# Autodesk Inventor assembly: GFRP_T2_18
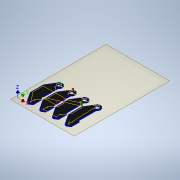
[picture p0: Inventor's stored thumbnail of the model, 180x180]
Saved by Autodesk Inventor 2020 (Build 240168000, 168)
## iProperties
Created: 2021-08-27
Part Number: GFRP_T2_18
Document SubType Name: Assembly
Designer: Masato
Author: Masato
## Documents named in this file (3)
- D:\GitHub\inventor\SUSTAINA-OP\Cam\GFRP_T2_18.iam
- D:\GitHub\inventor\SUSTAINA-OP\Cam\DisposableBoard.ipt
- D:\GitHub\inventor\SUSTAINA-OP\LowerBody\Link\FrontLink_frame.ipt
## Components (5 placed, 2 different names)
1. DisposableBoard:1 — メイト:2, メイト:1, フラッシュ:1, フラッシュ:2, メイト:6, メイト:7, 正接:2
2. FrontLink_frame:1 — メイト:6, メイト:7, 正接:2
3. FrontLink_frame:2
4. FrontLink_frame:3
5. FrontLink_frame:4
## Component patterns: (4 elements, first: FrontLink_frame:1)
## Relationships (7: Mate 4, Flush 2, Tangent 1)
- メイト:2 [Mate]: DisposableBoard:1
- メイト:1 [Mate]: DisposableBoard:1
- フラッシュ:1 [Flush]: DisposableBoard:1
- フラッシュ:2 [Flush]: DisposableBoard:1
- メイト:6 [Mate] (5 mm): DisposableBoard:1 ↔ FrontLink_frame:1
- メイト:7 [Mate]: DisposableBoard:1 ↔ FrontLink_frame:1
- 正接:2 [Tangent] (2 mm): DisposableBoard:1 ↔ FrontLink_frame:1
